# Autodesk Inventor assembly: Station Assembly
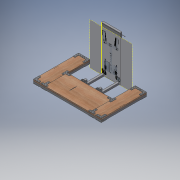
[picture p0: Inventor's stored thumbnail of the model, 180x180]
Saved by Autodesk Inventor 2018 (Build 220112000, 112)
## iProperties
Created: 2018-12-30
Part Number: Station Assembly
Document SubType Name: Assembly
Designer: maste
Author: maste
## Documents named in this file (11)
- C:\Users\maste\OneDrive\Documents\GitHub\2019CAD\Drive Station (Marching Band Edition)\Station Assembly.iam
- C:\Users\maste\OneDrive\Documents\GitHub\2019CAD\Drive Station (Marching Band Edition)\3ft 1x1.ipt
- C:\Users\maste\OneDrive\Documents\GitHub\2019CAD\Drive Station (Marching Band Edition)\2ft 1x1.ipt
- C:\Users\maste\OneDrive\Documents\GitHub\2019CAD\Drive Station (Marching Band Edition)\23in 1x1.ipt
- C:\Users\maste\OneDrive\Documents\GitHub\2019CAD\Drive Station (Marching Band Edition)\4in 1x1.ipt
- C:\Users\maste\OneDrive\Documents\GitHub\2019CAD\Drive Station (Marching Band Edition)\0.125 L-Gusset.ipt
- C:\Users\maste\OneDrive\Documents\GitHub\2019CAD\Drive Station (Marching Band Edition)\0.125 T-Gusset.ipt
- C:\Users\maste\OneDrive\Documents\GitHub\2019CAD\Drive Station (Marching Band Edition)\2in 1x2.ipt
- C:\Users\maste\OneDrive\Documents\GitHub\2019CAD\Drive Station (Marching Band Edition)\Middle Board.ipt
- C:\Users\maste\OneDrive\Documents\GitHub\2019CAD\Drive Station (Marching Band Edition)\Side Board.ipt
- C:\Users\maste\OneDrive\Documents\GitHub\2019CAD\Drive Station (Marching Band Edition)\Pretend this is a harness.ipt
## Components (34 placed, 10 different names)
1. 3ft 1x1:1 — Mate:1, Mate:2, Mate:3, Mate:10, Mate:11, Mate:12, Mate:65, Mate:66, Mate:75, Mate:76, Mate:77, Mate:82, Mate:84, Mate:89, Mate:90, Mate:91, Mate:106
2. 2ft 1x1:1 — Mate:45, Mate:46, Mate:48, Mate:50, Mate:93, Mate:94, Mate:95, Mate:96, Mate:97, Mate:98, Mate:105
3. 23in 1x1:1 — Mate:1, Mate:2, Mate:3, Mate:4, Mate:5, Mate:6, Mate:59, Mate:60, Mate:78
4. 23in 1x1:2 — Mate:10, Mate:11, Mate:12, Mate:13, Mate:14, Mate:15, Mate:41, Mate:42, Mate:43, Mate:92, Mate:101
5. 23in 1x1:3 — Mate:16, Mate:17, Mate:18, Mate:37, Mate:38, Mate:39, Mate:47, Mate:83, Mate:100
6. 23in 1x1:4 — Mate:7, Mate:8, Mate:9, Mate:49, Mate:62, Mate:63, Mate:67, Mate:104
7. 4in 1x1:1 — Mate:4, Mate:5, Mate:6, Mate:7, Mate:8, Mate:9, Mate:61, Mate:64, Mate:102, Mate:103
8. 4in 1x1:2 — Mate:13, Mate:14, Mate:15, Mate:16, Mate:17, Mate:18, Mate:40, Mate:44, Mate:99
9. 0.125 L-Gusset:2 — Mate:89, Mate:90, Mate:91, Mate:92
10. 0.125 L-Gusset:3 — Mate:75, Mate:76, Mate:77, Mate:78
11. 0.125 L-Gusset:5 — Mate:59, Mate:60, Mate:61
12. 0.125 L-Gusset:7 — Mate:37, Mate:38, Mate:39, Mate:40
13. 0.125 L-Gusset:9 — Mate:41, Mate:42, Mate:43, Mate:44
14. 0.125 L-Gusset:11 — Mate:62, Mate:63, Mate:64
15. 0.125 T-Gusset:2 — Mate:82, Mate:83, Mate:84
16. 0.125 T-Gusset:4 — Mate:65, Mate:66, Mate:67
17. 0.125 T-Gusset:6 — Mate:45, Mate:46, Mate:47
18. 0.125 T-Gusset:8 — Mate:48, Mate:49, Mate:50
19. 2in 1x2:1 — Mate:94, Mate:97, Mate:98
20. 2in 1x2:2 — Mate:93, Mate:95, Mate:96, Mate:138, Mate:139, Mate:140, Mate:141
21. Middle Board:1 — Mate:105, Mate:106, Mate:107, Mate:115, Mate:130, Mate:135, Mate:136
22. Side Board:1 — Mate:99, Mate:100, Mate:101, Mate:107, Mate:108, Mate:109, Mate:110, Mate:111, Mate:112, Mate:113, Mate:114, Mate:116, Mate:117, Mate:118, Mate:119, Mate:120, Mate:121, Mate:122
23. Side Board:2 — Mate:102, Mate:103, Mate:104, Mate:123, Mate:124, Mate:125, Mate:126, Mate:127, Mate:128, Mate:129, Mate:131, Mate:132, Mate:133, Mate:134, Mate:137
24. 0.125 L-Gusset:12 — Mate:117, Mate:118, Mate:119
25. 0.125 L-Gusset:13 — Mate:132, Mate:133, Mate:134
26. 0.125 L-Gusset:14 — Mate:126, Mate:127, Mate:128
27. 0.125 L-Gusset:15 — Mate:111, Mate:112, Mate:113
28. 0.125 L-Gusset:16 — Mate:108, Mate:109, Mate:110
29. 0.125 L-Gusset:17 — Mate:123, Mate:124, Mate:125
30. 0.125 T-Gusset:9 — Mate:114, Mate:115, Mate:116
31. 0.125 T-Gusset:10 — Mate:120, Mate:121, Mate:122
32. 0.125 T-Gusset:11 — Mate:135, Mate:136, Mate:137
33. 0.125 T-Gusset:12 — Mate:129, Mate:130, Mate:131
34. Pretend this is a harness:1 — Mate:138, Mate:139, Mate:140, Mate:141
## Relationships (101: Mate 101)
- Mate:1: 3ft 1x1:1 ↔ 23in 1x1:1
- Mate:2: 3ft 1x1:1 ↔ 23in 1x1:1
- Mate:3: 3ft 1x1:1 ↔ 23in 1x1:1
- Mate:4: 23in 1x1:1 ↔ 4in 1x1:1
- Mate:5: 23in 1x1:1 ↔ 4in 1x1:1
- Mate:6: 23in 1x1:1 ↔ 4in 1x1:1
- Mate:7: 23in 1x1:4 ↔ 4in 1x1:1
- Mate:8: 23in 1x1:4 ↔ 4in 1x1:1
- Mate:9: 23in 1x1:4 ↔ 4in 1x1:1
- Mate:10: 3ft 1x1:1 ↔ 23in 1x1:2
- Mate:11: 3ft 1x1:1 ↔ 23in 1x1:2
- Mate:12: 3ft 1x1:1 ↔ 23in 1x1:2
- Mate:13: 23in 1x1:2 ↔ 4in 1x1:2
- Mate:14: 23in 1x1:2 ↔ 4in 1x1:2
- Mate:15: 23in 1x1:2 ↔ 4in 1x1:2
- Mate:16: 23in 1x1:3 ↔ 4in 1x1:2
- Mate:17: 23in 1x1:3 ↔ 4in 1x1:2
- Mate:18: 23in 1x1:3 ↔ 4in 1x1:2
- Mate:37: 23in 1x1:3 ↔ 0.125 L-Gusset:7
- Mate:38: 23in 1x1:3 ↔ 0.125 L-Gusset:7
- Mate:39: 23in 1x1:3 ↔ 0.125 L-Gusset:7
- Mate:40: 4in 1x1:2 ↔ 0.125 L-Gusset:7
- Mate:41: 23in 1x1:2 ↔ 0.125 L-Gusset:9
- Mate:42: 23in 1x1:2 ↔ 0.125 L-Gusset:9
- Mate:43: 23in 1x1:2 ↔ 0.125 L-Gusset:9
- Mate:44: 4in 1x1:2 ↔ 0.125 L-Gusset:9
- Mate:45: 2ft 1x1:1 ↔ 0.125 T-Gusset:6
- Mate:46: 2ft 1x1:1 ↔ 0.125 T-Gusset:6
- Mate:47: 23in 1x1:3 ↔ 0.125 T-Gusset:6
- Mate:48: 2ft 1x1:1 ↔ 0.125 T-Gusset:8
- Mate:49: 23in 1x1:4 ↔ 0.125 T-Gusset:8
- Mate:50: 2ft 1x1:1 ↔ 0.125 T-Gusset:8
- Mate:59: 23in 1x1:1 ↔ 0.125 L-Gusset:5
- Mate:60: 23in 1x1:1 ↔ 0.125 L-Gusset:5
- Mate:61: 4in 1x1:1 ↔ 0.125 L-Gusset:5
- Mate:62: 23in 1x1:4 ↔ 0.125 L-Gusset:11
- Mate:63: 23in 1x1:4 ↔ 0.125 L-Gusset:11
- Mate:64: 4in 1x1:1 ↔ 0.125 L-Gusset:11
- Mate:65: 3ft 1x1:1 ↔ 0.125 T-Gusset:4
- Mate:66: 3ft 1x1:1 ↔ 0.125 T-Gusset:4
- Mate:67: 23in 1x1:4 ↔ 0.125 T-Gusset:4
- Mate:75: 3ft 1x1:1 ↔ 0.125 L-Gusset:3
- Mate:76: 3ft 1x1:1 ↔ 0.125 L-Gusset:3
- Mate:77: 3ft 1x1:1 ↔ 0.125 L-Gusset:3
- Mate:78: 23in 1x1:1 ↔ 0.125 L-Gusset:3
- Mate:82: 3ft 1x1:1 ↔ 0.125 T-Gusset:2
- Mate:83: 23in 1x1:3 ↔ 0.125 T-Gusset:2
- Mate:84: 3ft 1x1:1 ↔ 0.125 T-Gusset:2
- Mate:89: 3ft 1x1:1 ↔ 0.125 L-Gusset:2
- Mate:90: 3ft 1x1:1 ↔ 0.125 L-Gusset:2
- Mate:91: 3ft 1x1:1 ↔ 0.125 L-Gusset:2
- Mate:92: 23in 1x1:2 ↔ 0.125 L-Gusset:2
- Mate:93: 2ft 1x1:1 ↔ 2in 1x2:2
- Mate:94: 2ft 1x1:1 ↔ 2in 1x2:1
- Mate:95: 2ft 1x1:1 ↔ 2in 1x2:2
- Mate:96: 2ft 1x1:1 ↔ 2in 1x2:2
- Mate:97: 2ft 1x1:1 ↔ 2in 1x2:1
- Mate:98: 2ft 1x1:1 ↔ 2in 1x2:1
- Mate:99: 4in 1x1:2 ↔ Side Board:1
- Mate:100: 23in 1x1:3 ↔ Side Board:1
- Mate:101: 23in 1x1:2 ↔ Side Board:1
- Mate:102: 4in 1x1:1 ↔ Side Board:2
- Mate:103: 4in 1x1:1 ↔ Side Board:2
- Mate:104: 23in 1x1:4 ↔ Side Board:2
- Mate:105: 2ft 1x1:1 ↔ Middle Board:1
- Mate:106: 3ft 1x1:1 ↔ Middle Board:1
- Mate:107: Middle Board:1 ↔ Side Board:1
- Mate:108: Side Board:1 ↔ 0.125 L-Gusset:16
- Mate:109: Side Board:1 ↔ 0.125 L-Gusset:16
- Mate:110: Side Board:1 ↔ 0.125 L-Gusset:16
- Mate:111: Side Board:1 ↔ 0.125 L-Gusset:15
- Mate:112: Side Board:1 ↔ 0.125 L-Gusset:15
- Mate:113: Side Board:1 ↔ 0.125 L-Gusset:15
- Mate:114: Side Board:1 ↔ 0.125 T-Gusset:9
- Mate:115: Middle Board:1 ↔ 0.125 T-Gusset:9
- Mate:116: Side Board:1 ↔ 0.125 T-Gusset:9
- Mate:117: Side Board:1 ↔ 0.125 L-Gusset:12
- Mate:118: Side Board:1 ↔ 0.125 L-Gusset:12
- Mate:119: Side Board:1 ↔ 0.125 L-Gusset:12
- Mate:120: Side Board:1 ↔ 0.125 T-Gusset:10
- Mate:121: Side Board:1 ↔ 0.125 T-Gusset:10
- Mate:122: Side Board:1 ↔ 0.125 T-Gusset:10
- Mate:123: Side Board:2 ↔ 0.125 L-Gusset:17
- Mate:124: Side Board:2 ↔ 0.125 L-Gusset:17
- Mate:125: Side Board:2 ↔ 0.125 L-Gusset:17
- Mate:126: Side Board:2 ↔ 0.125 L-Gusset:14
- Mate:127: Side Board:2 ↔ 0.125 L-Gusset:14
- Mate:128: Side Board:2 ↔ 0.125 L-Gusset:14
- Mate:129: Side Board:2 ↔ 0.125 T-Gusset:12
- Mate:130: Middle Board:1 ↔ 0.125 T-Gusset:12
- Mate:131: Side Board:2 ↔ 0.125 T-Gusset:12
- Mate:132: Side Board:2 ↔ 0.125 L-Gusset:13
- Mate:133: Side Board:2 ↔ 0.125 L-Gusset:13
- Mate:134: Side Board:2 ↔ 0.125 L-Gusset:13
- Mate:135: Middle Board:1 ↔ 0.125 T-Gusset:11
- Mate:136: Middle Board:1 ↔ 0.125 T-Gusset:11
- Mate:137: Side Board:2 ↔ 0.125 T-Gusset:11
- Mate:138: 2in 1x2:2 ↔ Pretend this is a harness:1
- Mate:139: 2in 1x2:2 ↔ Pretend this is a harness:1
- Mate:140: 2in 1x2:2 ↔ Pretend this is a harness:1
- Mate:141: 2in 1x2:2 ↔ Pretend this is a harness:1
